# Autodesk Inventor assembly: rapoukLegAssemblyv0
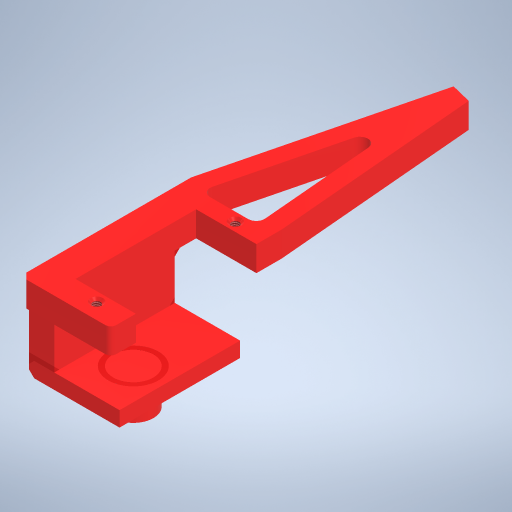
[picture p0: Inventor's stored thumbnail of the model, 512x512]
Saved by Autodesk Inventor 2024 (Build 280153000, 153)
## iProperties
Created: 2024-01-09
Part Number: rapoukLegAssemblyv0
Document SubType Name: Weldment
Designer: Roman Suk
Weld Material: Welded Aluminum-6061
Author: Roman Suk
## Documents named in this file (5)
- C:\Users\Roman Suk\Documents\Ročníkovka SŠ\CD\Technická dokumentace\rapoukLegAssemblyv0.iam
- C:\Users\Roman Suk\Documents\Ročníkovka SŠ\CD\Technická dokumentace\rapoukLegv9.ipt
- C:\Users\Roman Suk\Documents\Ročníkovka SŠ\CD\Technická dokumentace\rapoukLegSupportv2.ipt
- C:\Users\Roman Suk\Documents\Ročníkovka SŠ\CD\Technická dokumentace\rapoukLegBasev3.ipt
- C:\Users\Roman Suk\Documents\Ročníkovka SŠ\CD\Technická dokumentace\rapoukLegPinv1.ipt
## Components (4 placed, 4 different names)
1. rapoukLegv9:1 — Mate:1, Mate:2, Flush:1
2. rapoukLegSupportv2:1 — Mate:1, Mate:2, Flush:1, Mate:3, Flush:2, Flush:3
3. rapoukLegBasev3:1 — Mate:3, Flush:2, Flush:3, Flush:4, Tangent:1
4. rapoukLegPinv1:1 — Flush:4, Tangent:1
## Relationships (8: Flush 4, Mate 3, Tangent 1)
- Mate:1: rapoukLegv9:1 ↔ rapoukLegSupportv2:1
- Mate:2 (-3.25 mm): rapoukLegv9:1 ↔ rapoukLegSupportv2:1
- Flush:1: rapoukLegv9:1 ↔ rapoukLegSupportv2:1
- Mate:3: rapoukLegSupportv2:1 ↔ rapoukLegBasev3:1
- Flush:2: rapoukLegSupportv2:1 ↔ rapoukLegBasev3:1
- Flush:3: rapoukLegSupportv2:1 ↔ rapoukLegBasev3:1
- Flush:4: rapoukLegBasev3:1 ↔ rapoukLegPinv1:1
- Tangent:1: rapoukLegBasev3:1 ↔ rapoukLegPinv1:1
